# Autodesk Inventor assembly: wobble arm
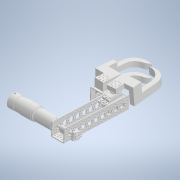
[picture p0: Inventor's stored thumbnail of the model, 180x180]
Saved by Autodesk Inventor 2021 (Build 250183000, 183)
## iProperties
Created: 2020-09-23
Part Number: wobble arm
Document SubType Name: Assembly
Designer: elois
Author: elois
## Documents named in this file (10)
- C:\Users\Owner\Documents\GitHub\CAD-2021-Ultimate_Goal\Wobble Goal\wobble arm.iam
- C:\Users\Owner\Documents\GitHub\CAD-2021-Ultimate_Goal\Wobble Goal\assembled servo block.iam
- C:\Users\Owner\Documents\GitHub\CAD-2021-Ultimate_Goal\Wobble Goal\wobble goal arm.ipt
- C:\Users\Owner\Documents\GitHub\CAD-2021-Ultimate_Goal\ServoCity\625051 assembly.ipt
- C:\Users\Owner\Documents\GitHub\CAD-2021-Ultimate_Goal\ServoCity\545588 assembly.ipt
- C:\Users\Owner\Documents\GitHub\CAD-2021-Ultimate_Goal\ServoCity\634158.ipt
- C:\Users\Owner\Documents\GitHub\CAD-2021-Ultimate_Goal\Wobble Goal\wobble goal arm_MIR1.ipt
- C:\Users\Owner\Documents\GitHub\CAD-2021-Ultimate_Goal\ServoCity\motor 188-1.ipt
- C:\Users\Owner\Documents\GitHub\CAD-2021-Ultimate_Goal\ServoCity\585440.ipt
- C:\Users\Owner\Documents\GitHub\CAD-2021-Ultimate_Goal\ServoCity\585448.ipt
## Components (9 placed, 9 different names)
1. assembled servo block:1 [sub-assembly] — Mate:19, Mate:20, Mate:27, Mate:28
2. motor 188-1:1 — Mate:10, Mate:11, Mate:23, Mate:24, Mate:26
3. wobble goal arm:1 — Mate:19, Mate:20
4. 585440:1 — Mate:29, Mate:30, Mate:31, Mate:32, Mate:33
5. 625051 assembly:1 — Mate:10, Mate:11, Mate:12, Mate:13, Mate:26
6. 545588 assembly:1 — Mate:14, Mate:15
7. 634158:1 — Mate:12, Mate:13, Mate:14, Mate:15, Mate:25
8. wobble goal arm_MIR1:1 — Mate:32, Mate:33
9. 585448:1 — Mate:23, Mate:24, Mate:25, Mate:27, Mate:28, Mate:29, Mate:30, Mate:31
## Relationships (19: Mate 19)
- Mate:10: motor 188-1:1 ↔ 625051 assembly:1
- Mate:11: motor 188-1:1 ↔ 625051 assembly:1
- Mate:12: 625051 assembly:1 ↔ 634158:1
- Mate:13: 625051 assembly:1 ↔ 634158:1
- Mate:14: 545588 assembly:1 ↔ 634158:1
- Mate:15: 545588 assembly:1 ↔ 634158:1
- Mate:19: assembled servo block:1 ↔ wobble goal arm:1
- Mate:20: assembled servo block:1 ↔ wobble goal arm:1
- Mate:23: motor 188-1:1 ↔ 585448:1
- Mate:24: motor 188-1:1 ↔ 585448:1
- Mate:25: 634158:1 ↔ 585448:1
- Mate:26: motor 188-1:1 ↔ 625051 assembly:1
- Mate:27: assembled servo block:1 ↔ 585448:1
- Mate:28: assembled servo block:1 ↔ 585448:1
- Mate:29: 585440:1 ↔ 585448:1
- Mate:30: 585440:1 ↔ 585448:1
- Mate:31: 585440:1 ↔ 585448:1
- Mate:32: 585440:1 ↔ wobble goal arm_MIR1:1
- Mate:33: 585440:1 ↔ wobble goal arm_MIR1:1
